# Autodesk Inventor assembly: Motors with Screws
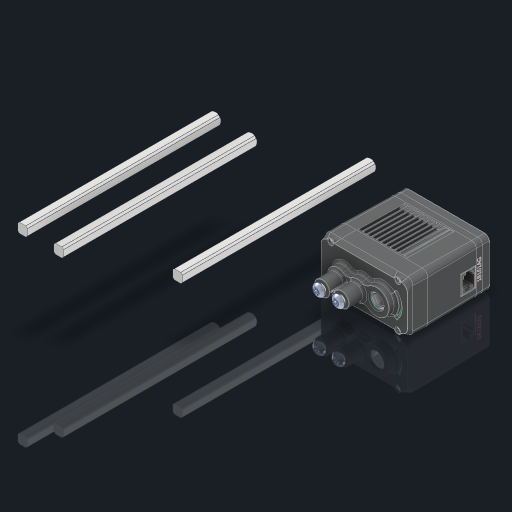
[picture p0: Inventor's stored thumbnail of the model, 512x512]
Saved by Autodesk Inventor 2023.2 (Build 272271030, 271C)
## iProperties
Created: 2022-08-18
Part Number: Motors with Screws
Document SubType Name: Assembly
Designer: ylu12
Author: ylu12
## Documents named in this file (14)
- C:\Users\black\OneDrive\Pictures\Documents\GitHub\New folder\2024-599Z\Cad\Library\VEX-CAD-Inventor-1.4.0\Electronics\Motors with Screws.iam
- C:\Users\black\OneDrive\Pictures\Documents\GitHub\New folder\2024-599Z\Cad\Library\VEX-CAD-Inventor-1.4.0\Electronics\V5 Motor.ipt
- C:\Users\black\OneDrive\Pictures\Documents\GitHub\New folder\2024-599Z\Cad\Library\VEX-CAD-Inventor-1.4.0\Structure\Hardware\Screw Steel - Hex\SScrew Hex Smooth .500.ipt
- C:\Users\ylu12\Documents\GitHub\VEX-CAD-Inventor\Structure\Hardware\Screw Steel - Hex.ipt
- C:\Users\black\OneDrive\Pictures\Documents\GitHub\New folder\2024-599Z\Cad\Library\VEX-CAD-Inventor-1.4.0\Structure\Hardware\Screw Steel - Star\SScrew Star Smooth .500.ipt
- C:\Users\ylu12\Documents\GitHub\VEX-CAD-Inventor\Structure\Hardware\Screw Steel - Star.ipt
- C:\Users\black\OneDrive\Pictures\Documents\GitHub\New folder\2024-599Z\Cad\Library\VEX-CAD-Inventor-1.4.0\Motion\Shaft HS\Shaft HS\Shaft HS 5.0 in.ipt
- C:\Users\black\OneDrive\Pictures\Documents\GitHub\New folder\2024-599Z\Cad\Library\VEX-CAD-Inventor-1.4.0\Motion\Shaft HS\Shaft HS.ipt
- C:\Users\black\OneDrive\Pictures\Documents\GitHub\New folder\2024-599Z\Cad\Shaft HS Part test\Shaft HS 5.0 in.ipt
- C:\Users\black\OneDrive\Pictures\Documents\GitHub\New folder\2024-599Z\Cad\Shaft HS Part test.ipt
- AluM-HexS.iam
- AluM-StarS.iam
- SteelM-HexS.iam
- SteelM-StarS.iam
## Components (8 placed, 4 different names)
1. V5 Motor:1 — Insert:1, Insert:2
2. SScrew Hex Smooth .500:1 — Insert:1, Insert:3
3. SScrew Hex Smooth .500:2 — Insert:2, Insert:4
4. SScrew Star Smooth .500:1 — Insert:4
5. SScrew Star Smooth .500:2 — Insert:3
6. Shaft HS 5.0 in:1
7. Shaft HS 5.0 in:2
8. Shaft HS 5.0 in:1
## Relationships (4: Insert 4)
- Insert:1 (1.5875 mm): V5 Motor:1 ↔ SScrew Hex Smooth .500:1
- Insert:2 (1.5875 mm): V5 Motor:1 ↔ SScrew Hex Smooth .500:2
- Insert:3: SScrew Hex Smooth .500:1 ↔ SScrew Star Smooth .500:2
- Insert:4: SScrew Hex Smooth .500:2 ↔ SScrew Star Smooth .500:1
## Named parameters: Thickness = 1.5875 mm
